# Autodesk Inventor assembly: Assembly-with-MCP3
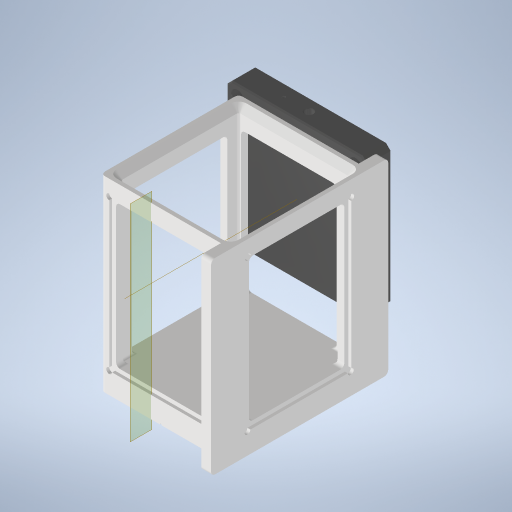
[picture p0: Inventor's stored thumbnail of the model, 512x512]
Saved by Autodesk Inventor 2024 (Build 280153000, 153)
## iProperties
Created: 2026-02-05
Part Number: Assembly-with-MCP3
Document SubType Name: Assembly
Designer: nvladi
Author: nvladi
## Documents named in this file (4)
- C:\Users\nvladi\Documents\GitHub\benchtop-hardware\Benchtop-CBI-Pittsburgh\custom_parts\ImmersionChambers\Slide-50x75mm-v1\Assembly-with-LCP03.iam
- Assembly-with-LCP03.iam
- C:\Users\nvladi\Documents\GitHub\benchtop-hardware\Benchtop-CBI-Pittsburgh\custom_parts\ImmersionChambers\Slide-50x75mm-v1\cuvette-w70mm-slide50x75mm-v2.ipt
- C:\Users\nvladi\Documents\GitHub\benchtop-hardware\Benchtop-2024(default-version)\CAD-model-Inventor\library\Thorlabs\60mm_cage_system\LCP03_M.ipt
## Components (2 placed, 2 different names)
1. cuvette-w70mm-slide50x75mm-v2:1 — Mate:2, Flush:1
2. LCP03_M:1 — Mate:1, Mate:2, Flush:1
## Relationships (3: Mate 2, Flush 1)
- Mate:1: LCP03_M:1
- Mate:2: cuvette-w70mm-slide50x75mm-v2:1 ↔ LCP03_M:1
- Flush:1: cuvette-w70mm-slide50x75mm-v2:1 ↔ LCP03_M:1
